# Autodesk Inventor assembly: SERVO
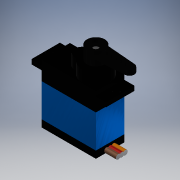
[picture p0: Inventor's stored thumbnail of the model, 180x180]
Saved by Autodesk Inventor 2017 (Build 210142000, 142)
## iProperties
Created: 2017-09-24
Part Number: SERVO
Document SubType Name: Assembly
Designer: Alexander Miller
Author: Alexander Miller
## Documents named in this file (3)
- C:\Users\Alexander Miller\Documents\Git\HeRo-Mini\Hardware\Assembly\SERVO.iam
- C:\Users\Alexander Miller\Documents\Git\HeRo-Mini\Hardware\Part\Misc\TP-MG92B.ipt
- C:\Users\Alexander Miller\Documents\Git\HeRo-Mini\Hardware\Part\Misc\TP-MG92B_HAT.ipt
## Components (2 placed, 2 different names)
1. TP-MG92B:1 — Rotational:1
2. TP-MG92B_HAT:1 — Rotational:1
## Relationships (1: RevoluteJoint 1)
- Rotational:1 [RevoluteJoint]: TP-MG92B:1 ↔ TP-MG92B_HAT:1
